# Autodesk Inventor assembly: Pushfit-Adapter_MIR_MIR2
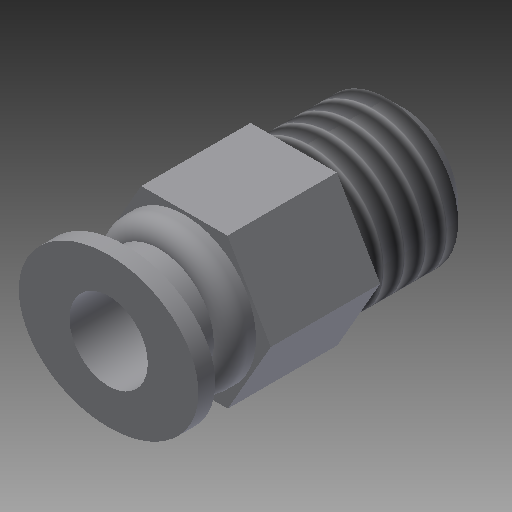
[picture p0: Inventor's stored thumbnail of the model, 512x512]
Saved by Autodesk Inventor 2017 (Build 210142000, 142)
## iProperties
Created: 2016-07-07
Part Number: Pushfit-Adapter_MIR_MIR2
Document SubType Name: Assembly
Designer: User
Author: joshmamo
## Documents named in this file (3)
- C:\All INVENTOR\SL-Inventor\SL-Beast 3D Printer\Pushfit-Adapter_MIR_MIR2.iam
- C:\All INVENTOR\SL-Inventor\SL-Beast 3D Printer\Pushfit-Adapter_MIR_MIR2.ipt
- C:\All INVENTOR\SL-Inventor\SL-Beast 3D Printer\Pushfit-adapter-cap_MIR_MIR2.ipt
## Components (2 placed, 2 different names)
1. Pushfit-Adapter_MIR_MIR2:1 — Flush:1
2. Pushfit-adapter-cap_MIR_MIR2:1 — Flush:1
## Relationships (1: Flush 1)
- Flush:1: Pushfit-Adapter_MIR_MIR2:1 ↔ Pushfit-adapter-cap_MIR_MIR2:1
